# Autodesk Inventor assembly: mg996r_right_mid_top_two_servo
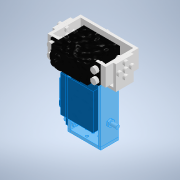
[picture p0: Inventor's stored thumbnail of the model, 180x180]
Saved by Autodesk Inventor 2021.4 (Build 254397000, 397)
## iProperties
Created: 2022-07-25
Part Number: mg996r_right_mid_top_two_servo
Document SubType Name: Assembly
Designer: isamu
Author: isamu
## Documents named in this file (3)
- D:\personal_projects\robot\inventor\2021_matlab_compat\mg996r_right_mid_top_two_servo.iam
- D:\personal_projects\robot\inventor\2021_matlab_compat\mg996r_bottom.iam
- D:\personal_projects\robot\inventor\2021_matlab_compat\mg996r_servo_frame_with_axis.iam
## Components (2 placed, 2 different names)
1. mg996r_bottom:1 [sub-assembly] — Mate:1, Mate:2, Mate:3
2. mg996r_servo_frame_with_axis:1 [sub-assembly] — Mate:1, Mate:2, Mate:3
## Relationships (3: Mate 3)
- Mate:1: mg996r_bottom:1 ↔ mg996r_servo_frame_with_axis:1
- Mate:2: mg996r_bottom:1 ↔ mg996r_servo_frame_with_axis:1
- Mate:3: mg996r_bottom:1 ↔ mg996r_servo_frame_with_axis:1
